# Autodesk Inventor assembly: print assembly 12.1
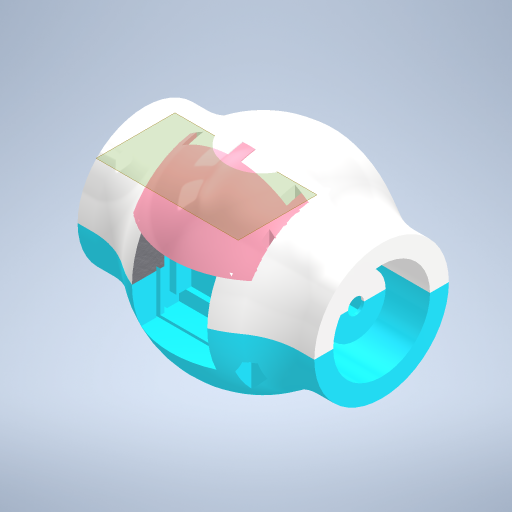
[picture p0: Inventor's stored thumbnail of the model, 512x512]
Saved by Autodesk Inventor 2023 (Build 270158000, 158)
## iProperties
Created: 2022-12-01
Part Number: print assembly 12.1
Document SubType Name: Assembly
Designer: RM206user
Author: RM206user
## Documents named in this file (4)
- C:\Users\RM206user\Desktop\cansat\tanekonsat2022_runback\machinary\assenbly\print assembly 12.1.iam
- C:\Users\RM206user\Desktop\cansat\tanekonsat2022_runback\machinary\body\body back\back moter middle tire ver\back moter middle lemon printing.ipt
- C:\Users\RM206user\Desktop\cansat\tanekonsat2022_runback\machinary\body\body back\back moter middle tire ver\back back printing pra.ipt
- C:\Users\RM206user\Desktop\cansat\tanekonsat2022_runback\machinary\body\body front\front lemon\body front moter middle lemon shape for printing.ipt
## Components (3 placed, 2 different names)
1. body moter middle:1 — メイト:1, メイト:2, メイト:3, メイト:5, メイト:6, メイト:7
2. body moter middle:2 — メイト:1, メイト:2, メイト:3
3. base front:1 — メイト:5, メイト:6, メイト:7
## Relationships (6: Mate 6)
- メイト:1 [Mate]: body moter middle:1 ↔ body moter middle:2
- メイト:2 [Mate]: body moter middle:1 ↔ body moter middle:2
- メイト:3 [Mate]: body moter middle:1 ↔ body moter middle:2
- メイト:5 [Mate]: body moter middle:1 ↔ base front:1
- メイト:6 [Mate]: body moter middle:1 ↔ base front:1
- メイト:7 [Mate]: body moter middle:1 ↔ base front:1
